# Autodesk Inventor assembly: manipulator_asembly
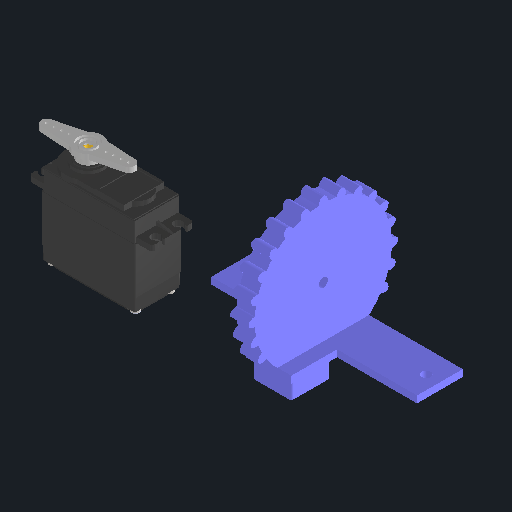
[picture p0: Inventor's stored thumbnail of the model, 512x512]
Saved by Autodesk Inventor 2024 (Build 280153000, 153)
## iProperties
Created: 2023-05-10
Part Number: manipulator_asembly
Document SubType Name: Assembly
Designer: user
Author: user
## Documents named in this file (3)
- D:\Docs\Robot\3d\machine_body\manipulator_asembly.iam
- D:\Docs\Robot\3d\machine_body\manipulator\bumper.ipt
- D:\Docs\Robot\3d\electronics\servo\MG996R SBORKA.iam
## Components (2 placed, 2 different names)
1. bumper:1 — Совмещение:1, Совмещение:2, Совмещение:3
2. MG996R SBORKA:1 [sub-assembly]
## Relationships (3: Mate 3)
- Совмещение:1 [Mate]: bumper:1
- Совмещение:2 [Mate]: bumper:1
- Совмещение:3 [Mate]: bumper:1
